# Autodesk Inventor assembly: rapoukBottomAssemblyv0
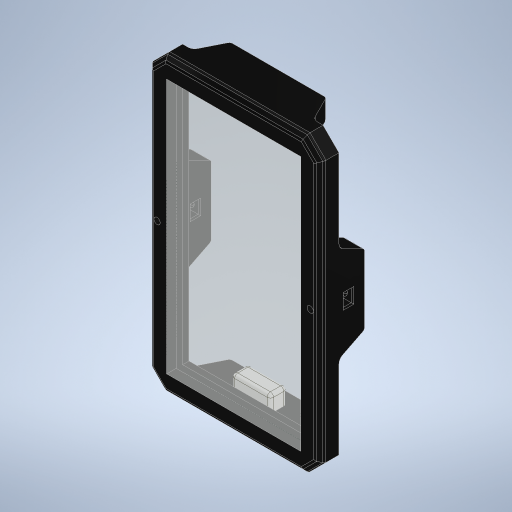
[picture p0: Inventor's stored thumbnail of the model, 512x512]
Saved by Autodesk Inventor 2024 (Build 280153000, 153)
## iProperties
Created: 2024-02-06
Part Number: rapoukBottomAssemblyv0
Document SubType Name: Weldment
Designer: Roman Suk
Weld Material: Welded Aluminum-6061
Author: Roman Suk
## Documents named in this file (4)
- C:\Users\Roman Suk\Documents\Ročníkovka SŠ\Technical documentation\Final1\rapoukBottomAssemblyv0.iam
- C:\Users\Roman Suk\Documents\Ročníkovka SŠ\Technical documentation\Final1\rapoukBottomCoverv0.ipt
- C:\Users\Roman Suk\Documents\Ročníkovka SŠ\Technical documentation\Final1\rapoukUSB-Cv0.ipt
- C:\Users\Roman Suk\Documents\Ročníkovka SŠ\Technical documentation\Final1\rapoukBottomPlexiv0.ipt
## Components (3 placed, 3 different names)
1. rapoukBottomCoverv0:1 — Mate:1, Mate:2, Mate:3, Mate:4, Mate:5, Mate:6
2. rapoukUSB-Cv0:1 — Mate:4, Mate:5, Mate:6
3. rapoukBottomPlexiv0:1 — Mate:1, Mate:2, Mate:3
## Relationships (6: Mate 6)
- Mate:1: rapoukBottomCoverv0:1 ↔ rapoukBottomPlexiv0:1
- Mate:2: rapoukBottomCoverv0:1 ↔ rapoukBottomPlexiv0:1
- Mate:3: rapoukBottomCoverv0:1 ↔ rapoukBottomPlexiv0:1
- Mate:4: rapoukBottomCoverv0:1 ↔ rapoukUSB-Cv0:1
- Mate:5: rapoukBottomCoverv0:1 ↔ rapoukUSB-Cv0:1
- Mate:6: rapoukBottomCoverv0:1 ↔ rapoukUSB-Cv0:1
